# Autodesk Inventor assembly: POM_T5_13
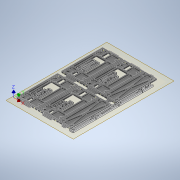
[picture p0: Inventor's stored thumbnail of the model, 180x180]
Saved by Autodesk Inventor 2022 (Build 260153000, 153)
## iProperties
Created: 2022-09-28
Part Number: POM_T5_13
Document SubType Name: Assembly
Designer: Masato
Author: Masato
## Documents named in this file (9)
- C:\Users\ヨコオリク\Documents\CITBrains\SUSTAINA-OP\Cam\POM_T5\POM_T5_13.iam
- C:\Users\ヨコオリク\Documents\CITBrains\SUSTAINA-OP\Cam\DisposableBoard.ipt
- C:\Users\ヨコオリク\Documents\CITBrains\SUSTAINA-OP\UpperBody\Cockpit\Cockpit_back_frame.ipt
- C:\Users\ヨコオリク\Documents\CITBrains\SUSTAINA-OP\UpperBody\Cockpit\Cockpit_battery_frame.ipt
- C:\Users\ヨコオリク\Documents\CITBrains\SUSTAINA-OP\OptionParts\DrillingJigs\Cockpit_back_frame_Jig.ipt
- C:\Users\ヨコオリク\Documents\CITBrains\SUSTAINA-OP\OptionParts\DrillingJigs\Cockpit_battery_back_door_Jig.ipt
- C:\Users\ヨコオリク\Documents\CITBrains\SUSTAINA-OP\OptionParts\DrillingJigs\Cockpit_battery_frame_Jig.ipt
- C:\Users\ヨコオリク\Documents\CITBrains\SUSTAINA-OP\OptionParts\DrillingJigs\Cockpit_front_frame_Jig.ipt
- C:\Users\ヨコオリク\Documents\CITBrains\SUSTAINA-OP\OptionParts\DrillingJigs\Cockpit_side_frame_Jig.ipt
## Components (19 placed, 8 different names)
1. DisposableBoard:1 — フラッシュ:1, フラッシュ:2, フラッシュ:3, フラッシュ:4, Flush:5, Flush:6, フラッシュ:7, フラッシュ:8
2. Cockpit_back_frame_Jig:1 — メイト:11, メイト:17, メイト:18, メイト:20
3. Cockpit_front_frame_Jig:1 — メイト:14, フラッシュ:7, メイト:16, メイト:17
4. Cockpit_front_frame_Jig:2 — メイト:19, メイト:20, メイト:21, メイト:29
5. Cockpit_battery_back_door_Jig:3 — メイト:24, メイト:25, メイト:26, メイト:32
6. Cockpit_battery_frame_Jig:3 — メイト:27, メイト:31, メイト:32
7. Cockpit_side_frame_Jig:3 — メイト:28, メイト:29, メイト:30
8. Cockpit_battery_frame:1 — Mate:4, メイト:15, フラッシュ:8, メイト:16, メイト:18
9. Cockpit_battery_frame:2 — メイト:21, メイト:30
10. Cockpit_back_frame:1 — Mate:1, Flush:5, Flush:6, メイト:6, メイト:7, メイト:10
11. Cockpit_back_frame:2 — メイト:15
12. Cockpit_back_frame:3 — メイト:22, メイト:23
13. Cockpit_back_frame:4 — メイト:25, メイト:26, メイト:31
14. Cockpit_battery_frame_Jig:1 — メイト:8, メイト:9, メイト:10
15. Cockpit_side_frame_Jig:1 — メイト:5, メイト:6, メイト:7, メイト:9
16. Cockpit_battery_frame_Jig:2
17. Cockpit_side_frame_Jig:2
18. Cockpit_battery_back_door_Jig:1 — メイト:12
19. Cockpit_battery_back_door_Jig:2 — メイト:22, メイト:23
## Component patterns: (2 elements, first: Cockpit_battery_frame:1), (4 elements, first: Cockpit_back_frame:1), (2 elements, first: Cockpit_battery_frame_Jig:1 + Cockpit_side_frame_Jig:1), (2 elements, first: Cockpit_battery_back_door_Jig:1)
## Relationships (37: Mate 29, Flush 8)
- フラッシュ:1 [Flush]: DisposableBoard:1
- フラッシュ:2 [Flush]: DisposableBoard:1
- フラッシュ:3 [Flush]: DisposableBoard:1
- フラッシュ:4 [Flush]: DisposableBoard:1
- Mate:1: Cockpit_back_frame:1
- Flush:5 (-2 mm): DisposableBoard:1 ↔ Cockpit_back_frame:1
- Flush:6 (-2 mm): DisposableBoard:1 ↔ Cockpit_back_frame:1
- Mate:4: Cockpit_battery_frame:1
- メイト:5 [Mate]: Cockpit_side_frame_Jig:1
- メイト:6 [Mate] (2.5 mm): Cockpit_back_frame:1 ↔ Cockpit_side_frame_Jig:1
- メイト:7 [Mate] (2.5 mm): Cockpit_back_frame:1 ↔ Cockpit_side_frame_Jig:1
- メイト:8 [Mate]: Cockpit_battery_frame_Jig:1
- メイト:9 [Mate] (2.1 mm): Cockpit_battery_frame_Jig:1 ↔ Cockpit_side_frame_Jig:1
- メイト:10 [Mate] (2.1 mm): Cockpit_back_frame:1 ↔ Cockpit_battery_frame_Jig:1
- メイト:11 [Mate]: Cockpit_back_frame_Jig:1
- メイト:12 [Mate]: Cockpit_battery_back_door_Jig:1
- メイト:14 [Mate]: Cockpit_front_frame_Jig:1
- フラッシュ:7 [Flush] (2 mm): DisposableBoard:1 ↔ Cockpit_front_frame_Jig:1
- メイト:15 [Mate] (2.1 mm): Cockpit_battery_frame:1 ↔ Cockpit_back_frame:2
- フラッシュ:8 [Flush] (-2.1 mm): DisposableBoard:1 ↔ Cockpit_battery_frame:1
- メイト:16 [Mate] (2.1 mm): Cockpit_front_frame_Jig:1 ↔ Cockpit_battery_frame:1
- メイト:17 [Mate] (2.1 mm): Cockpit_back_frame_Jig:1 ↔ Cockpit_front_frame_Jig:1
- メイト:18 [Mate] (2.1 mm): Cockpit_back_frame_Jig:1 ↔ Cockpit_battery_frame:1
- メイト:19 [Mate]: Cockpit_front_frame_Jig:2
- メイト:20 [Mate] (2.1 mm): Cockpit_back_frame_Jig:1 ↔ Cockpit_front_frame_Jig:2
- メイト:21 [Mate] (2.1 mm): Cockpit_front_frame_Jig:2 ↔ Cockpit_battery_frame:2
- メイト:22 [Mate] (2.5 mm): Cockpit_back_frame:3 ↔ Cockpit_battery_back_door_Jig:2
- メイト:23 [Mate] (2.5 mm): Cockpit_back_frame:3 ↔ Cockpit_battery_back_door_Jig:2
- メイト:24 [Mate]: Cockpit_battery_back_door_Jig:3
- メイト:25 [Mate] (2.5 mm): Cockpit_battery_back_door_Jig:3 ↔ Cockpit_back_frame:4
- メイト:26 [Mate] (2.5 mm): Cockpit_battery_back_door_Jig:3 ↔ Cockpit_back_frame:4
- メイト:27 [Mate]: Cockpit_battery_frame_Jig:3
- メイト:28 [Mate]: Cockpit_side_frame_Jig:3
- メイト:29 [Mate] (2.1 mm): Cockpit_front_frame_Jig:2 ↔ Cockpit_side_frame_Jig:3
- メイト:30 [Mate] (2.1 mm): Cockpit_side_frame_Jig:3 ↔ Cockpit_battery_frame:2
- メイト:31 [Mate] (2.5 mm): Cockpit_battery_frame_Jig:3 ↔ Cockpit_back_frame:4
- メイト:32 [Mate] (2.5 mm): Cockpit_battery_back_door_Jig:3 ↔ Cockpit_battery_frame_Jig:3
